# Autodesk Inventor assembly: Simulation_module_2
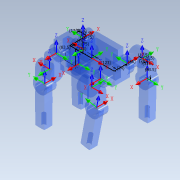
[picture p0: Inventor's stored thumbnail of the model, 180x180]
Saved by Autodesk Inventor 2020 (Build 240168000, 168)
## iProperties
Created: 2021-01-12
Part Number: Simulation_module_2
Document SubType Name: Assembly
Designer: DELL
Author: DELL
## Documents named in this file (6)
- F:\SoftRobot2.0\FlexipodFast\mesh\v5.0\Simulation_module.iam
- F:\SoftRobot2.0\FlexipodFast\mesh\v5.0\body.ipt
- F:\SoftRobot2.0\FlexipodFast\mesh\v5.0\hip.ipt
- F:\SoftRobot2.0\FlexipodFast\mesh\v5.0\hip_back.ipt
- F:\SoftRobot2.0\FlexipodFast\mesh\v5.0\thigh.ipt
- F:\SoftRobot2.0\FlexipodFast\mesh\v5.0\shank.ipt
## Components (13 placed, 5 different names)
1. body:1 — Mate:1, Mate:2, Flush:1, Flush:2, Flush:3, Angle:1, Angle:2, Mate:7, Mate:8, Angle:4, Angle:5, Mate:13, Mate:14, Angle:7, Mate:15, Mate:16, Angle:8
2. hip:3 — Mate:1, Mate:2, Angle:1, Mate:3, Mate:4
3. hip:4 — Mate:7, Mate:8, Angle:4, Mate:9, Mate:10
4. thigh:7 — Mate:3, Mate:4, Angle:2, Mate:6, Flush:4, Mate:25
5. thigh:8 — Mate:9, Mate:10, Angle:5, Mate:12, Flush:8
6. shank:7 — Mate:12, Flush:8
7. shank:6 — Mate:6, Flush:5, Mate:25
8. hip_back:2 — Mate:13, Mate:14, Angle:7, Mate:17, Mate:18, Angle:9, Flush:7
9. hip_back:1 — Mate:15, Mate:16, Angle:8, Mate:19, Mate:20, Angle:10
10. thigh:9 — Mate:17, Mate:18, Angle:9, Mate:24, Flush:9
11. thigh:10 — Mate:19, Mate:20, Angle:10, Mate:22, Mate:26
12. shank:5 — Mate:22, Mate:26
13. shank:4 — Mate:24, Flush:6, Flush:9
## Relationships (39: Mate 22, Flush 9, Angle 8)
- Mate:1: body:1 ↔ hip:3
- Mate:2: body:1 ↔ hip:3
- Flush:1: body:1
- Flush:2: body:1
- Flush:3: body:1
- Angle:1 (0 deg): body:1 ↔ hip:3
- Mate:3 (-10.5 mm): hip:3 ↔ thigh:7
- Mate:4: hip:3 ↔ thigh:7
- Angle:2 (0 deg): body:1 ↔ thigh:7
- Mate:6: thigh:7 ↔ shank:6
- Mate:7: body:1 ↔ hip:4
- Mate:8: body:1 ↔ hip:4
- Angle:4 (0 deg): body:1 ↔ hip:4
- Mate:9 (-10.5 mm): hip:4 ↔ thigh:8
- Mate:10: hip:4 ↔ thigh:8
- Angle:5 (0 deg): body:1 ↔ thigh:8
- Mate:12: thigh:8 ↔ shank:7
- Mate:13: body:1 ↔ hip_back:2
- Mate:14: body:1 ↔ hip_back:2
- Angle:7 (0 deg): body:1 ↔ hip_back:2
- Mate:15: body:1 ↔ hip_back:1
- Mate:16: body:1 ↔ hip_back:1
- Angle:8 (0 deg): body:1 ↔ hip_back:1
- Mate:17 (-9 mm): hip_back:2 ↔ thigh:9
- Mate:18: hip_back:2 ↔ thigh:9
- Angle:9 (0 deg): hip_back:2 ↔ thigh:9
- Mate:19 (-9 mm): hip_back:1 ↔ thigh:10
- Mate:20: hip_back:1 ↔ thigh:10
- Angle:10 (0 deg): hip_back:1 ↔ thigh:10
- Mate:22: thigh:10 ↔ shank:5
- Mate:24: thigh:9 ↔ shank:4
- Flush:4: thigh:7
- Flush:5: shank:6
- Flush:6: shank:4
- Flush:7: hip_back:2
- Flush:8: thigh:8 ↔ shank:7
- Mate:25: thigh:7 ↔ shank:6
- Flush:9: thigh:9 ↔ shank:4
- Mate:26: thigh:10 ↔ shank:5
